# Autodesk Inventor assembly: folivora
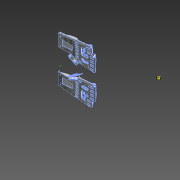
[picture p0: Inventor's stored thumbnail of the model, 180x180]
Saved by Autodesk Inventor 2018 (Build 220112000, 112)
## iProperties
Created: 2018-05-16
Part Number: folivora
Material: 一般
Document SubType Name: Assembly
Designer: NaMACHAN
Mass: 511.38 g
Surface Area: 1744.23 cm^2
Volume: 200.35 cm^3
Density: 2.55243 g/cm^3
Author: NaMACHAN
## Documents named in this file (28)
- C:\Users\NaMACHAN\Dropbox\Project\original\folivora\inventor\folivora.iam
- C:\Users\NaMACHAN\Dropbox\Project\original\folivora\inventor\baseframe.ipt
- C:\Users\NaMACHAN\Dropbox\Project\original\folivora\inventor\keyplate4.ipt
- C:\Users\NaMACHAN\Dropbox\Project\original\folivora\inventor\ball.ipt
- C:\Users\NaMACHAN\Dropbox\Project\original\folivora\inventor\trackball-base.ipt
- C:\Users\NaMACHAN\Dropbox\Project\original\folivora\inventor\trackball-shaft.ipt
- C:\Users\NaMACHAN\Dropbox\Project\original\folivora\inventor\bearing.ipt
- C:\Users\NaMACHAN\Dropbox\Project\original\folivora\inventor\bearingcover.ipt
- C:\Users\NaMACHAN\Dropbox\Project\original\folivora\inventor\trackball_l.ipt
- C:\Users\NaMACHAN\Dropbox\Project\original\folivora\inventor\trackball-cover.ipt
- C:\Users\NaMACHAN\Dropbox\Project\original\folivora\inventor\trackball-spacer.ipt
- C:\Users\NaMACHAN\Dropbox\Project\original\folivora\inventor\keyplate5.ipt
- C:\Users\NaMACHAN\Dropbox\Project\original\folivora\inventor\drawings\spacer-c1-near.ipt
- C:\Users\NaMACHAN\Dropbox\Project\original\folivora\inventor\drawings\spacer-c1-far.ipt
- C:\Users\NaMACHAN\Dropbox\Project\original\folivora\inventor\drawings\spacer-c2-far.ipt
- C:\Users\NaMACHAN\Dropbox\Project\original\folivora\inventor\drawings\spacer-c2-near.ipt
- C:\Users\NaMACHAN\Dropbox\Project\original\folivora\inventor\baseframe_left.ipt
- C:\Users\NaMACHAN\Dropbox\Project\original\folivora\inventor\keyplate2.ipt
- C:\Users\NaMACHAN\Dropbox\Project\original\folivora\inventor\drawings\thumbkey-base.ipt
- C:\Users\NaMACHAN\Dropbox\Project\original\folivora\inventor\drawings\ristrest.ipt
- C:\Users\NaMACHAN\Dropbox\Project\original\folivora\inventor\palmrest.ipt
- C:\Users\NaMACHAN\Dropbox\Project\original\folivora\inventor\palmrest_left.ipt
- C:\Users\NaMACHAN\Dropbox\Project\original\folivora\inventor\folivora\AIP\FEA\cjjue1qww.fins
- C:\Users\NaMACHAN\Dropbox\Project\original\folivora\inventor\folivora\AIP\FEA\cjjue1qww.fsat
- C:\Users\NaMACHAN\Dropbox\Project\original\folivora\inventor\folivora\AIP\FEA\cjjue1qww.ftes
- C:\Users\NaMACHAN\Dropbox\Project\original\folivora\inventor\folivora\AIP\FEA\cjjue1qww.fwiz
- C:\Users\NaMACHAN\Dropbox\Project\original\folivora\inventor\folivora\AIP\FEA\cjjue1r1c.fmsh
- C:\Users\NaMACHAN\Dropbox\Project\original\folivora\inventor\folivora\AIP\FEA\cjjue1r1d.fres
## Components (88 placed, 21 different names)
1. ball:1 — メイト:105, メイト:115
2. trackball-base:1 — メイト:52, メイト:53, メイト:54, メイト:55, メイト:56, メイト:57, メイト:58, メイト:59, メイト:60, メイト:61, メイト:62, メイト:63, フラッシュ:15, メイト:105, フラッシュ:16, メイト:117, メイト:118, メイト:119, メイト:120, メイト:124, メイト:125
3. trackball-shaft:1 — メイト:49, メイト:52, メイト:53, メイト:54
4. bearing:1 — メイト:49, メイト:55
5. trackball-shaft:2 — メイト:56, メイト:57, メイト:59
6. bearing:2 — メイト:58
7. trackball-shaft:3 — メイト:60, メイト:61, メイト:62
8. bearing:3 — メイト:63
9. bearingcover:1 — フラッシュ:15, フラッシュ:16, メイト:115, メイト:121, メイト:122, メイト:123, メイト:124, メイト:125, メイト:134, メイト:135, メイト:136
10. trackball_l:1 — メイト:121, メイト:122, メイト:123, メイト:245, フラッシュ:21, フラッシュ:22
11. trackball-shaft:4 — メイト:116, メイト:117, メイト:118, メイト:119
12. bearing:4 — メイト:116, メイト:120
13. trackball-cover:1 — メイト:126, メイト:127, メイト:128, メイト:129, メイト:130, メイト:131, メイト:132, メイト:133
14. trackball-spacer:1 — メイト:126, メイト:130, メイト:136
15. trackball-spacer:2 — メイト:129, メイト:131, メイト:135
16. trackball-spacer:3 — メイト:128, メイト:133
17. trackball-spacer:4 — メイト:127, メイト:132, メイト:134
18. baseframe:1 — メイト:147, メイト:154, メイト:160, メイト:161, メイト:162, メイト:163, メイト:188, メイト:189, メイト:194, メイト:198, メイト:199, メイト:200, メイト:209, メイト:210, メイト:219, メイト:220, メイト:221, メイト:222, メイト:223, メイト:224, メイト:225, メイト:226, メイト:227, メイト:228, フラッシュ:19, フラッシュ:20, メイト:230, メイト:245, フラッシュ:21, フラッシュ:22, メイト:323, フラッシュ:24, メイト:324
19. keyplate4:1 — メイト:137, メイト:138, メイト:139, メイト:140, メイト:141, メイト:143, メイト:144, メイト:159
20. spacer-c1-near:1 — メイト:137, メイト:139, メイト:147
21. spacer-c1-near:2 — メイト:138, メイト:140
22. spacer-c1-far:1 — メイト:141, メイト:143, メイト:163, メイト:226
23. spacer-c1-far:2 — メイト:144, メイト:159, メイト:162
24. keyplate5:1 — メイト:148, メイト:149, メイト:150, メイト:151, メイト:155, メイト:156, メイト:157, メイト:158
25. spacer-c2-far:1 — メイト:148, メイト:150, メイト:154, メイト:160
26. spacer-c2-far:2 — メイト:149, メイト:151, メイト:161, メイト:224
27. spacer-c2-near:1 — メイト:155, メイト:157
28. spacer-c2-near:2 — メイト:156, メイト:158
29. keyplate5:2
30. spacer-c2-far:3 — メイト:188, メイト:194
31. spacer-c2-far:4 — メイト:189, メイト:225
32. spacer-c2-near:3
33. spacer-c2-near:4
34. keyplate5:4
35. spacer-c2-far:7 — メイト:200
36. spacer-c2-far:8 — メイト:199
37. spacer-c2-near:7 — メイト:198
38. spacer-c2-near:8 — メイト:223
39. keyplate4:2
40. spacer-c1-near:3
41. spacer-c1-near:4 — メイト:221
42. spacer-c1-far:3 — メイト:210, メイト:227
43. spacer-c1-far:4 — メイト:209
44. keyplate4:3
45. spacer-c1-near:5 — メイト:222
46. spacer-c1-near:6
47. spacer-c1-far:5 — メイト:220, メイト:228
48. spacer-c1-far:6 — メイト:219
49. baseframe_left:1 — フラッシュ:19, フラッシュ:20, メイト:230, メイト:246, フラッシュ:23, メイト:256, メイト:273, メイト:274, メイト:275, メイト:276, メイト:277, メイト:278, メイト:279, メイト:280, メイト:289, メイト:290, メイト:291, メイト:292, メイト:293, メイト:294, メイト:296, メイト:313, メイト:314, メイト:315, メイト:316, メイト:317, メイト:318, メイト:319, メイト:320, フラッシュ:25, メイト:325, メイト:326
50. keyplate2:1 — メイト:234, メイト:236, メイト:239, メイト:240, メイト:241, メイト:242, メイト:243, メイト:244
51. thumbkey-base:1 — メイト:232, メイト:233, メイト:235, メイト:246, フラッシュ:23
52. spacer-c1-near:7 — メイト:232, メイト:233, メイト:234, メイト:239
53. spacer-c1-near:8 — メイト:235, メイト:236, メイト:240
54. spacer-c1-near:9 — メイト:241, メイト:244
55. spacer-c1-near:10 — メイト:242, メイト:243
56. keyplate4:4 — メイト:295
57. spacer-c1-near:11
58. spacer-c1-near:12
59. spacer-c1-far:7 — メイト:293, メイト:295, メイト:296
60. spacer-c1-far:8 — メイト:256, メイト:294
61. keyplate4:5
62. spacer-c1-near:13
63. spacer-c1-near:14
64. spacer-c1-far:9 — メイト:278
65. spacer-c1-far:10 — メイト:274, メイト:279, メイト:280
66. keyplate4:6
67. spacer-c1-near:15
68. spacer-c1-near:16 — メイト:276
69. spacer-c1-far:11 — メイト:273, メイト:277
70. spacer-c1-far:12 — メイト:275
71. keyplate5:5
72. spacer-c2-far:9 — メイト:290, メイト:291, メイト:292
73. spacer-c2-far:10 — メイト:289
74. spacer-c2-near:9
75. spacer-c2-near:10
76. keyplate5:6
77. spacer-c2-far:11 — メイト:313, メイト:316
78. spacer-c2-far:12 — メイト:315, メイト:317
79. spacer-c2-near:11
80. spacer-c2-near:12
81. keyplate5:7
82. spacer-c2-far:13 — メイト:314, メイト:319
83. spacer-c2-far:14 — メイト:318, メイト:320
84. spacer-c2-near:13
85. spacer-c2-near:14
86. ristrest:1
87. palmrest:1 — メイト:323, フラッシュ:24, メイト:324
88. palmrest_left:1 — フラッシュ:25, メイト:325, メイト:326
## Relationships (209: Mate 200, Flush 9)
- メイト:49 [Mate]: trackball-shaft:1 ↔ bearing:1
- [Mate]: trackball-shaft:2 ↔ bearing:2
- [Mate]: trackball-shaft:3 ↔ bearing:3
- メイト:52 [Mate] (1.5 mm): trackball-base:1 ↔ trackball-shaft:1
- メイト:53 [Mate] (1.5 mm): trackball-base:1 ↔ trackball-shaft:1
- メイト:54 [Mate]: trackball-base:1 ↔ trackball-shaft:1
- メイト:55 [Mate] (0.5 mm): trackball-base:1 ↔ bearing:1
- メイト:56 [Mate] (1.5 mm): trackball-base:1 ↔ trackball-shaft:2
- メイト:57 [Mate] (1.5 mm): trackball-base:1 ↔ trackball-shaft:2
- メイト:58 [Mate] (0.5 mm): trackball-base:1 ↔ bearing:2
- メイト:59 [Mate]: trackball-base:1 ↔ trackball-shaft:2
- メイト:60 [Mate] (1.5 mm): trackball-base:1 ↔ trackball-shaft:3
- メイト:61 [Mate] (1.5 mm): trackball-base:1 ↔ trackball-shaft:3
- メイト:62 [Mate]: trackball-base:1 ↔ trackball-shaft:3
- メイト:63 [Mate] (0.5 mm): trackball-base:1 ↔ bearing:3
- フラッシュ:15 [Flush]: trackball-base:1 ↔ bearingcover:1
- メイト:105 [Mate]: ball:1 ↔ trackball-base:1
- フラッシュ:16 [Flush]: trackball-base:1 ↔ bearingcover:1
- メイト:115 [Mate] (6.4 mm): ball:1 ↔ bearingcover:1
- メイト:116 [Mate]: trackball-shaft:4 ↔ bearing:4
- メイト:117 [Mate] (1.5 mm): trackball-base:1 ↔ trackball-shaft:4
- メイト:118 [Mate] (1.5 mm): trackball-base:1 ↔ trackball-shaft:4
- メイト:119 [Mate]: trackball-base:1 ↔ trackball-shaft:4
- メイト:120 [Mate] (0.5 mm): trackball-base:1 ↔ bearing:4
- メイト:121 [Mate]: bearingcover:1 ↔ trackball_l:1
- メイト:122 [Mate]: bearingcover:1 ↔ trackball_l:1
- メイト:123 [Mate]: bearingcover:1 ↔ trackball_l:1
- メイト:124 [Mate]: trackball-base:1 ↔ bearingcover:1
- メイト:125 [Mate]: trackball-base:1 ↔ bearingcover:1
- メイト:126 [Mate]: trackball-cover:1 ↔ trackball-spacer:1
- メイト:127 [Mate]: trackball-cover:1 ↔ trackball-spacer:4
- メイト:128 [Mate]: trackball-cover:1 ↔ trackball-spacer:3
- メイト:129 [Mate]: trackball-cover:1 ↔ trackball-spacer:2
- メイト:130 [Mate]: trackball-cover:1 ↔ trackball-spacer:1
- メイト:131 [Mate]: trackball-cover:1 ↔ trackball-spacer:2
- メイト:132 [Mate]: trackball-cover:1 ↔ trackball-spacer:4
- メイト:133 [Mate]: trackball-cover:1 ↔ trackball-spacer:3
- メイト:134 [Mate]: bearingcover:1 ↔ trackball-spacer:4
- メイト:135 [Mate]: bearingcover:1 ↔ trackball-spacer:2
- メイト:136 [Mate]: bearingcover:1 ↔ trackball-spacer:1
- メイト:137 [Mate]: keyplate4:1 ↔ spacer-c1-near:1
- メイト:138 [Mate]: keyplate4:1 ↔ spacer-c1-near:2
- メイト:139 [Mate]: keyplate4:1 ↔ spacer-c1-near:1
- メイト:140 [Mate]: keyplate4:1 ↔ spacer-c1-near:2
- メイト:141 [Mate]: keyplate4:1 ↔ spacer-c1-far:1
- メイト:143 [Mate]: keyplate4:1 ↔ spacer-c1-far:1
- メイト:144 [Mate]: keyplate4:1 ↔ spacer-c1-far:2
- メイト:147 [Mate]: baseframe:1 ↔ spacer-c1-near:1
- メイト:148 [Mate]: keyplate5:1 ↔ spacer-c2-far:1
- メイト:149 [Mate]: keyplate5:1 ↔ spacer-c2-far:2
- メイト:150 [Mate]: keyplate5:1 ↔ spacer-c2-far:1
- メイト:151 [Mate]: keyplate5:1 ↔ spacer-c2-far:2
- メイト:154 [Mate]: baseframe:1 ↔ spacer-c2-far:1
- メイト:155 [Mate]: keyplate5:1 ↔ spacer-c2-near:1
- メイト:156 [Mate]: keyplate5:1 ↔ spacer-c2-near:2
- メイト:157 [Mate]: keyplate5:1 ↔ spacer-c2-near:1
- メイト:158 [Mate]: keyplate5:1 ↔ spacer-c2-near:2
- メイト:159 [Mate]: keyplate4:1 ↔ spacer-c1-far:2
- メイト:160 [Mate] (1.5 mm): baseframe:1 ↔ spacer-c2-far:1
- メイト:161 [Mate] (1.5 mm): baseframe:1 ↔ spacer-c2-far:2
- メイト:162 [Mate] (1.5 mm): baseframe:1 ↔ spacer-c1-far:2
- メイト:163 [Mate] (1.5 mm): baseframe:1 ↔ spacer-c1-far:1
- [Mate]: keyplate5:2 ↔ spacer-c2-far:3
- [Mate]: keyplate5:2 ↔ spacer-c2-far:4
- [Mate]: keyplate5:2 ↔ spacer-c2-far:3
- [Mate]: keyplate5:2 ↔ spacer-c2-far:4
- [Mate]: keyplate5:2 ↔ spacer-c2-near:3
- [Mate]: keyplate5:2 ↔ spacer-c2-near:4
- [Mate]: keyplate5:2 ↔ spacer-c2-near:3
- [Mate]: keyplate5:2 ↔ spacer-c2-near:4
- [Mate]: keyplate5:4 ↔ spacer-c2-far:7
- [Mate]: keyplate5:4 ↔ spacer-c2-far:8
- [Mate]: keyplate5:4 ↔ spacer-c2-far:7
- [Mate]: keyplate5:4 ↔ spacer-c2-far:8
- [Mate]: keyplate5:4 ↔ spacer-c2-near:7
- [Mate]: keyplate5:4 ↔ spacer-c2-near:8
- [Mate]: keyplate5:4 ↔ spacer-c2-near:7
- [Mate]: keyplate5:4 ↔ spacer-c2-near:8
- メイト:188 [Mate] (1.5 mm): baseframe:1 ↔ spacer-c2-far:3
- メイト:189 [Mate] (1.5 mm): baseframe:1 ↔ spacer-c2-far:4
- メイト:194 [Mate]: baseframe:1 ↔ spacer-c2-far:3
- メイト:198 [Mate]: baseframe:1 ↔ spacer-c2-near:7
- メイト:199 [Mate] (1.5 mm): baseframe:1 ↔ spacer-c2-far:8
- メイト:200 [Mate] (1.5 mm): baseframe:1 ↔ spacer-c2-far:7
- [Mate]: keyplate4:2 ↔ spacer-c1-near:3
- [Mate]: keyplate4:2 ↔ spacer-c1-near:4
- [Mate]: keyplate4:2 ↔ spacer-c1-near:3
- [Mate]: keyplate4:2 ↔ spacer-c1-near:4
- [Mate]: keyplate4:2 ↔ spacer-c1-far:3
- [Mate]: keyplate4:2 ↔ spacer-c1-far:3
- [Mate]: keyplate4:2 ↔ spacer-c1-far:4
- [Mate]: keyplate4:2 ↔ spacer-c1-far:4
- メイト:209 [Mate] (1.5 mm): baseframe:1 ↔ spacer-c1-far:4
- メイト:210 [Mate] (1.5 mm): baseframe:1 ↔ spacer-c1-far:3
- [Mate]: keyplate4:3 ↔ spacer-c1-near:5
- [Mate]: keyplate4:3 ↔ spacer-c1-near:6
- [Mate]: keyplate4:3 ↔ spacer-c1-near:5
- [Mate]: keyplate4:3 ↔ spacer-c1-near:6
- [Mate]: keyplate4:3 ↔ spacer-c1-far:5
- [Mate]: keyplate4:3 ↔ spacer-c1-far:5
- [Mate]: keyplate4:3 ↔ spacer-c1-far:6
- [Mate]: keyplate4:3 ↔ spacer-c1-far:6
- メイト:219 [Mate] (1.5 mm): baseframe:1 ↔ spacer-c1-far:6
- メイト:220 [Mate] (1.5 mm): baseframe:1 ↔ spacer-c1-far:5
- メイト:221 [Mate]: baseframe:1 ↔ spacer-c1-near:4
- メイト:222 [Mate]: baseframe:1 ↔ spacer-c1-near:5
- メイト:223 [Mate] (-20 mm): baseframe:1 ↔ spacer-c2-near:8
- メイト:224 [Mate] (-18 mm): baseframe:1 ↔ spacer-c2-far:2
- メイト:225 [Mate] (-20 mm): baseframe:1 ↔ spacer-c2-far:4
- メイト:226 [Mate] (-22 mm): baseframe:1 ↔ spacer-c1-far:1
- メイト:227 [Mate] (-20 mm): baseframe:1 ↔ spacer-c1-far:3
- メイト:228 [Mate] (-21 mm): baseframe:1 ↔ spacer-c1-far:5
- フラッシュ:19 [Flush]: baseframe:1 ↔ baseframe_left:1
- フラッシュ:20 [Flush]: baseframe:1 ↔ baseframe_left:1
- メイト:230 [Mate] (150 mm): baseframe:1 ↔ baseframe_left:1
- メイト:232 [Mate]: thumbkey-base:1 ↔ spacer-c1-near:7
- メイト:233 [Mate]: thumbkey-base:1 ↔ spacer-c1-near:7
- メイト:234 [Mate]: keyplate2:1 ↔ spacer-c1-near:7
- メイト:235 [Mate]: thumbkey-base:1 ↔ spacer-c1-near:8
- メイト:236 [Mate]: keyplate2:1 ↔ spacer-c1-near:8
- メイト:239 [Mate]: keyplate2:1 ↔ spacer-c1-near:7
- メイト:240 [Mate]: keyplate2:1 ↔ spacer-c1-near:8
- メイト:241 [Mate]: keyplate2:1 ↔ spacer-c1-near:9
- メイト:242 [Mate]: keyplate2:1 ↔ spacer-c1-near:10
- メイト:243 [Mate]: keyplate2:1 ↔ spacer-c1-near:10
- メイト:244 [Mate]: keyplate2:1 ↔ spacer-c1-near:9
- メイト:245 [Mate]: trackball_l:1 ↔ baseframe:1
- フラッシュ:21 [Flush] (-8 mm): trackball_l:1 ↔ baseframe:1
- フラッシュ:22 [Flush]: trackball_l:1 ↔ baseframe:1
- メイト:246 [Mate]: baseframe_left:1 ↔ thumbkey-base:1
- フラッシュ:23 [Flush]: baseframe_left:1 ↔ thumbkey-base:1
- [Mate]: keyplate4:4 ↔ spacer-c1-near:11
- [Mate]: keyplate4:4 ↔ spacer-c1-near:12
- [Mate]: keyplate4:4 ↔ spacer-c1-near:11
- [Mate]: keyplate4:4 ↔ spacer-c1-near:12
- [Mate]: keyplate4:4 ↔ spacer-c1-far:7
- [Mate]: keyplate4:4 ↔ spacer-c1-far:8
- [Mate]: keyplate4:4 ↔ spacer-c1-far:8
- メイト:256 [Mate]: baseframe_left:1 ↔ spacer-c1-far:8
- [Mate]: keyplate4:5 ↔ spacer-c1-near:13
- [Mate]: keyplate4:5 ↔ spacer-c1-near:14
- [Mate]: keyplate4:5 ↔ spacer-c1-near:13
- [Mate]: keyplate4:5 ↔ spacer-c1-near:14
- [Mate]: keyplate4:5 ↔ spacer-c1-far:9
- [Mate]: keyplate4:5 ↔ spacer-c1-far:9
- [Mate]: keyplate4:5 ↔ spacer-c1-far:10
- [Mate]: keyplate4:5 ↔ spacer-c1-far:10
- [Mate]: keyplate4:6 ↔ spacer-c1-near:15
- [Mate]: keyplate4:6 ↔ spacer-c1-near:16
- [Mate]: keyplate4:6 ↔ spacer-c1-near:15
- [Mate]: keyplate4:6 ↔ spacer-c1-near:16
- [Mate]: keyplate4:6 ↔ spacer-c1-far:11
- [Mate]: keyplate4:6 ↔ spacer-c1-far:11
- [Mate]: keyplate4:6 ↔ spacer-c1-far:12
- [Mate]: keyplate4:6 ↔ spacer-c1-far:12
- メイト:273 [Mate]: baseframe_left:1 ↔ spacer-c1-far:11
- メイト:274 [Mate]: baseframe_left:1 ↔ spacer-c1-far:10
- メイト:275 [Mate] (1.5 mm): baseframe_left:1 ↔ spacer-c1-far:12
- メイト:276 [Mate] (1.5 mm): baseframe_left:1 ↔ spacer-c1-near:16
- メイト:277 [Mate] (-15 mm): baseframe_left:1 ↔ spacer-c1-far:11
- メイト:278 [Mate] (1.5 mm): baseframe_left:1 ↔ spacer-c1-far:9
- メイト:279 [Mate] (1.5 mm): baseframe_left:1 ↔ spacer-c1-far:10
- メイト:280 [Mate] (-13 mm): baseframe_left:1 ↔ spacer-c1-far:10
- [Mate]: keyplate5:5 ↔ spacer-c2-far:9
- [Mate]: keyplate5:5 ↔ spacer-c2-far:10
- [Mate]: keyplate5:5 ↔ spacer-c2-far:9
- [Mate]: keyplate5:5 ↔ spacer-c2-far:10
- [Mate]: keyplate5:5 ↔ spacer-c2-near:9
- [Mate]: keyplate5:5 ↔ spacer-c2-near:10
- [Mate]: keyplate5:5 ↔ spacer-c2-near:9
- [Mate]: keyplate5:5 ↔ spacer-c2-near:10
- メイト:289 [Mate]: baseframe_left:1 ↔ spacer-c2-far:10
- メイト:290 [Mate]: baseframe_left:1 ↔ spacer-c2-far:9
- メイト:291 [Mate]: baseframe_left:1 ↔ spacer-c2-far:9
- メイト:292 [Mate] (-18 mm): baseframe_left:1 ↔ spacer-c2-far:9
- メイト:293 [Mate] (1.5 mm): baseframe_left:1 ↔ spacer-c1-far:7
- メイト:294 [Mate] (1.5 mm): baseframe_left:1 ↔ spacer-c1-far:8
- メイト:295 [Mate]: keyplate4:4 ↔ spacer-c1-far:7
- メイト:296 [Mate] (-20 mm): baseframe_left:1 ↔ spacer-c1-far:7
- [Mate]: keyplate5:6 ↔ spacer-c2-far:11
- [Mate]: keyplate5:6 ↔ spacer-c2-far:12
- [Mate]: keyplate5:6 ↔ spacer-c2-far:11
- [Mate]: keyplate5:6 ↔ spacer-c2-far:12
- [Mate]: keyplate5:6 ↔ spacer-c2-near:11
- [Mate]: keyplate5:6 ↔ spacer-c2-near:12
- [Mate]: keyplate5:6 ↔ spacer-c2-near:11
- [Mate]: keyplate5:6 ↔ spacer-c2-near:12
- [Mate]: keyplate5:7 ↔ spacer-c2-far:13
- [Mate]: keyplate5:7 ↔ spacer-c2-far:14
- [Mate]: keyplate5:7 ↔ spacer-c2-far:13
- [Mate]: keyplate5:7 ↔ spacer-c2-far:14
- [Mate]: keyplate5:7 ↔ spacer-c2-near:13
- [Mate]: keyplate5:7 ↔ spacer-c2-near:14
- [Mate]: keyplate5:7 ↔ spacer-c2-near:13
- [Mate]: keyplate5:7 ↔ spacer-c2-near:14
- メイト:313 [Mate]: baseframe_left:1 ↔ spacer-c2-far:11
- メイト:314 [Mate]: baseframe_left:1 ↔ spacer-c2-far:13
- メイト:315 [Mate] (1.5 mm): baseframe_left:1 ↔ spacer-c2-far:12
- メイト:316 [Mate] (1.5 mm): baseframe_left:1 ↔ spacer-c2-far:11
- メイト:317 [Mate] (-16 mm): baseframe_left:1 ↔ spacer-c2-far:12
- メイト:318 [Mate] (1.5 mm): baseframe_left:1 ↔ spacer-c2-far:14
- メイト:319 [Mate] (1.5 mm): baseframe_left:1 ↔ spacer-c2-far:13
- メイト:320 [Mate] (-19 mm): baseframe_left:1 ↔ spacer-c2-far:14
- メイト:323 [Mate]: baseframe:1 ↔ palmrest:1
- フラッシュ:24 [Flush] (8 mm): baseframe:1 ↔ palmrest:1
- メイト:324 [Mate] (-110 mm): baseframe:1 ↔ palmrest:1
- フラッシュ:25 [Flush] (8 mm): baseframe_left:1 ↔ palmrest_left:1
- メイト:325 [Mate]: baseframe_left:1 ↔ palmrest_left:1
- メイト:326 [Mate] (-110 mm): baseframe_left:1 ↔ palmrest_left:1
## Named parameters: sa_0 = 7.4e-12, sa_1 = -5000, sa_2 = 4e-13, sa_3 = -1.32e-11, sa_4 = -5000, sa_5 = -4.2e-12, sa_6 = -2.8e-12, sa_7 = -5000, sa_8 = -2.3e-12, sa_9 = -1e-12, sa_10 = -5000, sa_11 = -3.7e-12, sa_12 = 2.78e-11, sa_13 = -5000, sa_14 = 7e-12, sa_15 = 1.85e-11, sa_16 = -5000, sa_17 = 3.9e-12, d430_d429 = 0 mm, d431_d429 = 0 mm, d959_d943 = 0 mm, d960_d944 = 0 mm, d961_d945 = 0 mm, d962_d946 = 0 mm, d963_d950 = 0 mm, d964_d951 = 0 mm, d965_d952 = 0 mm, d966_d953 = 0 mm, d975_d943 = 0 mm, d976_d944 = 0 mm, d977_d945 = 0 mm, d978_d946 = 0 mm, d979_d950 = 0 mm, d980_d951 = 0 mm, d981_d952 = 0 mm, d982_d953 = 0 mm, d1004_d933 = 0 mm, d1005_d934 = 0 mm, d1006_d935 = 0 mm, d1007_d937 = 0 mm, d1008_d938 = 0 mm, d1009_d954 = 0 mm, d1010_d931 = 0 mm, d1011_d932 = 0 mm, d1014_d933 = 0 mm, d1015_d934 = 0 mm, d1016_d935 = 0 mm, d1017_d937 = 0 mm, d1018_d938 = 0 mm, d1019_d954 = 0 mm, d1020_d931 = 0 mm, d1021_d932 = 0 mm, d1075_d933 = 0 mm, d1076_d934 = 0 mm, d1078_d937 = 0 mm, d1079_d938 = 0 mm, d1080_d954 = 0 mm, d1081_d931 = 0 mm, d1082_d932 = 0 mm, d1085_d933 = 0 mm, d1086_d934 = 0 mm, d1087_d935 = 0 mm, d1088_d937 = 0 mm, d1089_d938 = 0 mm, d1090_d954 = 0 mm, d1091_d931 = 0 mm, d1092_d932 = 0 mm, d1093_d933 = 0 mm, d1094_d934 = 0 mm, d1095_d935 = 0 mm, d1096_d937 = 0 mm, d1097_d938 = 0 mm, d1098_d954 = 0 mm, d1099_d931 = 0 mm, d1100_d932 = 0 mm, d1109_d959_d943 = 0 mm, d1110_d960_d944 = 0 mm, d1111_d961_d945 = 0 mm, d1112_d962_d946 = 0 mm, d1113_d963_d950 = 0 mm, d1114_d964_d951 = 0 mm, d1115_d965_d952 = 0 mm, d1116_d966_d953 = 0 mm, d1125_d959_d943 = 0 mm, d1126_d960_d944 = 0 mm, d1127_d961_d945 = 0 mm, d1128_d962_d946 = 0 mm, d1129_d963_d950 = 0 mm, d1130_d964_d951 = 0 mm, d1131_d965_d952 = 0 mm, d1132_d966_d953 = 0 mm, d1133_d959_d943 = 0 mm, d1134_d960_d944 = 0 mm, d1135_d961_d945 = 0 mm, d1136_d962_d946 = 0 mm, d1137_d963_d950 = 0 mm, d1138_d964_d951 = 0 mm, d1139_d965_d952 = 0 mm, d1140_d966_d953 = 0 mm
note: some values were not read from the file. Shown as the stored number, unit unknown: "sa_0", "sa_1", "sa_2", "sa_3", "sa_4", "sa_5", "sa_6", "sa_7", "sa_8", "sa_9", "sa_10", "sa_11", "sa_12", "sa_13", "sa_14", "sa_15", "sa_16", "sa_17".
